# Autodesk Inventor assembly: Baugruppe1
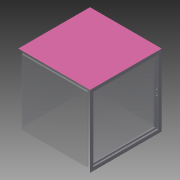
[picture p0: Inventor's stored thumbnail of the model, 180x180]
Saved by Autodesk Inventor 2018.2 (Build 222227000, 227)
## iProperties
Created: 2019-09-20
Part Number: Baugruppe1
Material: Generisch
Document SubType Name: Assembly
Designer: Lolob
Author: Lolob
## Documents named in this file (7)
- C:\Users\Lolob\Documents\Dipl\Smartcube_Construction\Version_3\Baugruppe1.iam
- C:\Users\Lolob\Documents\Dipl\Smartcube_Construction\Version_2\PV_Modul.ipt
- C:\Users\Lolob\Documents\Dipl\Smartcube_Construction\Version_2\PV_Modul_CPY.ipt
- C:\Users\Lolob\Documents\Dipl\Smartcube_Construction\Version_2\PV_Ramen_CPY_3.ipt
- C:\Users\Lolob\Documents\Dipl\Smartcube_Construction\Version_2\PV_Modul_CPY_3.ipt
- C:\Users\Lolob\Documents\Dipl\Smartcube_Construction\Version_2\PV_Modul_CPY_3_3.ipt
- C:\Users\Lolob\Documents\Dipl\Smartcube_Construction\Version_3\Boden.ipt
## Components (6 placed, 6 different names)
1. Boden:1
2. PV_Modul:1
3. PV_Modul_CPY:1
4. PV_Ramen_CPY_3:1 — Starr:4, Passend:5, Passend:6, Fluchtend:1
5. PV_Modul_CPY_3:1 — Starr:4
6. PV_Modul_CPY_3_3:1
## Relationships (4: Mate 2, WeldJoint 1, Flush 1)
- Starr:4 [WeldJoint]: PV_Ramen_CPY_3:1 ↔ PV_Modul_CPY_3:1
- Passend:5 [Mate]: PV_Ramen_CPY_3:1
- Passend:6 [Mate]: PV_Ramen_CPY_3:1
- Fluchtend:1 [Flush]: PV_Ramen_CPY_3:1
